# Autodesk Inventor assembly: floor
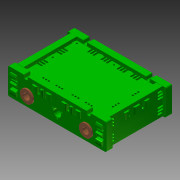
[picture p0: Inventor's stored thumbnail of the model, 180x180]
Saved by Autodesk Inventor 2012 SP1 (Build 160190100, 190)
## iProperties
Created: 2011-11-06
Part Number: floor
Document SubType Name: Assembly
Designer: Aaron
Author: Aaron
## Documents named in this file (7)
- C:\Users\Aaron\Documents\Projects\MTM-Snap-Metric\floor.iam
- C:\Users\Aaron\Documents\Projects\MTM-Snap-Metric\floor_base.ipt
- C:\Users\Aaron\Documents\Projects\MTM-Snap-Metric\floor_back.ipt
- C:\Users\Aaron\Documents\Projects\MTM-Snap-Metric\floor_front.ipt
- C:\Users\Aaron\Documents\Projects\MTM-Snap-Metric\floor_sideA.ipt
- C:\Users\Aaron\Documents\Projects\MTM-Snap-Metric\floor_sideB.ipt
- C:\Users\Aaron\Documents\Projects\InventorParts\Bearing\SHFZ12_25.ipt
## Components (9 placed, 6 different names)
1. floor_base:1 — Mate:1, Mate:2, Mate:3, Mate:4, Mate:5, Mate:6, Mate:7, Mate:8, Mate:9, Mate:10, Mate:11, Mate:12
2. floor_back:1 — Mate:1, Mate:2, Mate:3
3. floor_front:1 — Mate:4, Mate:5, Mate:6
4. floor_sideA:1 — Mate:7, Mate:8, Mate:9, Insert:3, Insert:4
5. floor_sideB:1 — Mate:10, Mate:11, Mate:12, Insert:1, Insert:2
6. SHFZ12-25:1 — Insert:1
7. SHFZ12-25:2 — Insert:2
8. SHFZ12-25:3 — Insert:3
9. SHFZ12-25:4 — Insert:4
## Relationships (16: Mate 12, Insert 4)
- Mate:1: floor_base:1 ↔ floor_back:1
- Mate:2: floor_base:1 ↔ floor_back:1
- Mate:3: floor_base:1 ↔ floor_back:1
- Mate:4: floor_base:1 ↔ floor_front:1
- Mate:5: floor_base:1 ↔ floor_front:1
- Mate:6: floor_base:1 ↔ floor_front:1
- Mate:7: floor_base:1 ↔ floor_sideA:1
- Mate:8: floor_base:1 ↔ floor_sideA:1
- Mate:9: floor_base:1 ↔ floor_sideA:1
- Mate:10: floor_base:1 ↔ floor_sideB:1
- Mate:11: floor_base:1 ↔ floor_sideB:1
- Mate:12: floor_base:1 ↔ floor_sideB:1
- Insert:1: floor_sideB:1 ↔ SHFZ12-25:1
- Insert:2: floor_sideB:1 ↔ SHFZ12-25:2
- Insert:3: floor_sideA:1 ↔ SHFZ12-25:3
- Insert:4: floor_sideA:1 ↔ SHFZ12-25:4
